# Autodesk Inventor assembly: Drivebox
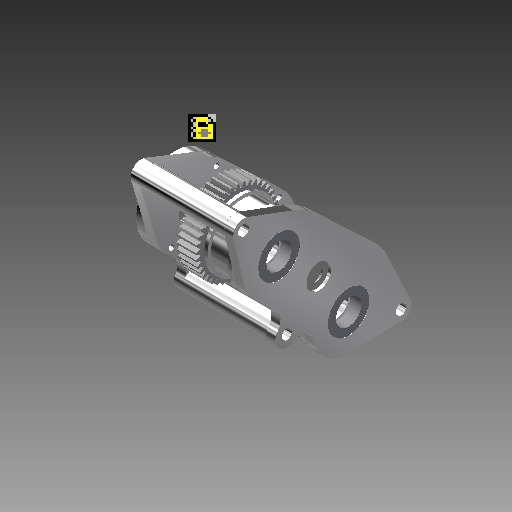
[picture p0: Inventor's stored thumbnail of the model, 512x512]
Saved by Autodesk Inventor 2019.4 (Build 234330000, 330)
## iProperties
Created: 2020-01-05
Part Number: Drivebox
Document SubType Name: Assembly
Designer: Mark
Mass: 1259.7 g
Surface Area: 1353.8 cm^2
Volume: 329.953 cm^3
Density: 3.8178 g/cm^3
Author: Mark
## Documents named in this file (13)
- C:\Users\Mark\Desktop\7738 Helion Engineering\7738-2020\CAD\Gearbox\Drivebox.iam
- C:\Users\Mark\Desktop\7738 Helion Engineering\7738-2020\CAD\Gearbox\Gearbox Plate 1.ipt
- C:\Users\Mark\Desktop\7738 Helion Engineering\7738-2020\CAD\Gearbox\Gearbox Plate 2.ipt
- C:\Users\Mark\Desktop\7738 Helion Engineering\7738-2020\CAD\Gearbox\Shaft Jr.ipt
- C:\Users\Mark\Desktop\7738 Helion Engineering\7738-2020\CAD\Gearbox\F6800.ipt
- C:\Users\Mark\Desktop\7738 Helion Engineering\7738-2020\CAD\Gearbox\Spacer.ipt
- C:\Users\Mark\Desktop\7738 Helion Engineering\7738-2020\CAD\Gearbox\F6804.ipt
- C:\Users\Mark\Desktop\7738 Helion Engineering\7738-2020\CAD\Gearbox\10T_Steel_Spur_Gear_20_DP_12T_Center_Distance_Falcon_Motor_217-6917.ipt
- C:\Users\Mark\Desktop\7738 Helion Engineering\7738-2020\CAD\Gearbox\40t_Aluminum_Spur_Gear_20_DP_1_2_Hex_Bore_217-2708.ipt
- C:\Users\Mark\Desktop\7738 Helion Engineering\7738-2020\CAD\Gearbox\Gearbox\Design Accelerator\Spur Gears1.iam
- C:\Users\Mark\Desktop\7738 Helion Engineering\7738-2020\CAD\Gearbox\Gearbox\Design Accelerator\Spur Gears2.iam
- C:\Users\Mark\Desktop\7738 Helion Engineering\7738-2020\CAD\Gearbox\HTD 5M 30 20mm ID Keyed.ipt
- C:\Users\Mark\Desktop\7738 Helion Engineering\7738-2020\CAD\Motor Spacer.ipt
## Components (19 placed, 11 different names)
1. Gearbox Plate 1:1 — Mate:3, Mate:4, Mate:13, Mate:14, Mate:25, Mate:26, Flush:3, Mate:43, Mate:45, Mate:46, Mate:47, Mate:54, Mate:56
2. Gearbox Plate 2:1 — Mate:33, Mate:34, Mate:35, Mate:36, Mate:37, Mate:38, Mate:39, Flush:3, Mate:40, Mate:49, Mate:51, Mate:44
3. Shaft Jr:1 — Mate:7, Mate:8, Mate:41
4. F6800:1 — Mate:3, Mate:4, Mate:7, Mate:8, Mate:39, Mate:42
5. F6800:2 — Mate:37, Mate:38, Mate:41
6. Spacer:1 — Mate:44, Mate:45
7. Spacer:2 — Mate:46, Mate:47
8. Spacer:3 — Mate:13, Mate:14
9. F6804:1 — Mate:31, Mate:33, Mate:34, Mate:50
10. F6804:2 — Mate:32, Mate:35, Mate:36, Mate:48
11. 10T_Steel_Spur_Gear_20_DP_12T_Center_Distance_Falcon_Motor_217-6917:1 — Mate:25
12. 10T_Steel_Spur_Gear_20_DP_12T_Center_Distance_Falcon_Motor_217-6917:2 — Mate:26
13. 40t_Aluminum_Spur_Gear_20_DP_1_2_Hex_Bore_217-2708:1 — Mate:30, Mate:42, Mate:43
14. Spur Gears:1 [sub-assembly] — Mate:30, Mate:31, Flush:2, Mate:40
15. Spur Gears:2 [sub-assembly] — Mate:32, Flush:2
16. HTD 5M 30 20mm ID Keyed:2 — Mate:48, Mate:49
17. HTD 5M 30 20mm ID Keyed:3 — Mate:50, Mate:51
18. Motor Spacer:1 — Mate:54
19. Motor Spacer:2 — Mate:56
## Relationships (34: Mate 32, Flush 2)
- Mate:3: Gearbox Plate 1:1 ↔ F6800:1
- Mate:4: Gearbox Plate 1:1 ↔ F6800:1
- Mate:7: Shaft Jr:1 ↔ F6800:1
- Mate:8 (0.2 mm): Shaft Jr:1 ↔ F6800:1
- Mate:13: Gearbox Plate 1:1 ↔ Spacer:3
- Mate:14: Gearbox Plate 1:1 ↔ Spacer:3
- Mate:25 (1 mm): Gearbox Plate 1:1 ↔ 10T_Steel_Spur_Gear_20_DP_12T_Center_Distance_Falcon_Motor_217-6917:1
- Mate:26 (1 mm): Gearbox Plate 1:1 ↔ 10T_Steel_Spur_Gear_20_DP_12T_Center_Distance_Falcon_Motor_217-6917:2
- Mate:30 (8 mm): 40t_Aluminum_Spur_Gear_20_DP_1_2_Hex_Bore_217-2708:1 ↔ Spur Gears:1
- Mate:31: F6804:1 ↔ Spur Gears:1
- Mate:32: F6804:2 ↔ Spur Gears:2
- Flush:2: Spur Gears:1 ↔ Spur Gears:2
- Mate:33: Gearbox Plate 2:1 ↔ F6804:1
- Mate:34: Gearbox Plate 2:1 ↔ F6804:1
- Mate:35: Gearbox Plate 2:1 ↔ F6804:2
- Mate:36: Gearbox Plate 2:1 ↔ F6804:2
- Mate:37: Gearbox Plate 2:1 ↔ F6800:2
- Mate:38: Gearbox Plate 2:1 ↔ F6800:2
- Mate:39: Gearbox Plate 2:1 ↔ F6800:1
- Flush:3: Gearbox Plate 1:1 ↔ Gearbox Plate 2:1
- Mate:40: Gearbox Plate 2:1 ↔ Spur Gears:1
- Mate:41 (0.2 mm): Shaft Jr:1 ↔ F6800:2
- Mate:42: F6800:1 ↔ 40t_Aluminum_Spur_Gear_20_DP_1_2_Hex_Bore_217-2708:1
- Mate:43 (4 mm): Gearbox Plate 1:1 ↔ 40t_Aluminum_Spur_Gear_20_DP_1_2_Hex_Bore_217-2708:1
- Mate:44: Gearbox Plate 2:1 ↔ Spacer:1
- Mate:45: Gearbox Plate 1:1 ↔ Spacer:1
- Mate:46: Gearbox Plate 1:1 ↔ Spacer:2
- Mate:47: Gearbox Plate 1:1 ↔ Spacer:2
- Mate:48: F6804:2 ↔ HTD 5M 30 20mm ID Keyed:2
- Mate:49 (3 mm): Gearbox Plate 2:1 ↔ HTD 5M 30 20mm ID Keyed:2
- Mate:50: F6804:1 ↔ HTD 5M 30 20mm ID Keyed:3
- Mate:51 (3 mm): Gearbox Plate 2:1 ↔ HTD 5M 30 20mm ID Keyed:3
- Mate:54: Gearbox Plate 1:1 ↔ Motor Spacer:1
- Mate:56: Gearbox Plate 1:1 ↔ Motor Spacer:2
